# Autodesk Inventor assembly: EncoderAssembly_MIR1
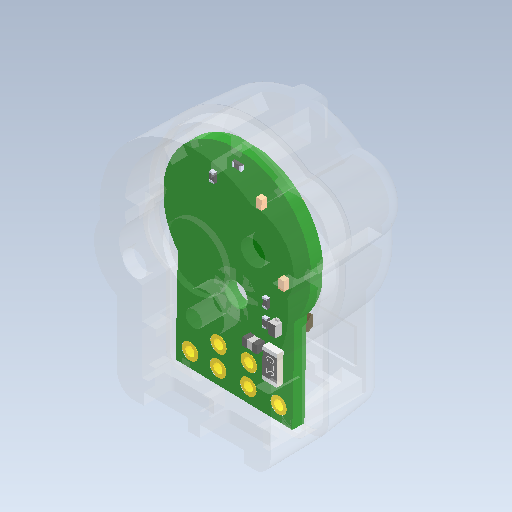
[picture p0: Inventor's stored thumbnail of the model, 512x512]
Saved by Autodesk Inventor 2020 (Build 240168000, 168)
## iProperties
Created: 2021-02-20
Part Number: EncoderAssembly_MIR1
Document SubType Name: Assembly
Designer: turnm
Author: turnm
## Documents named in this file (3)
- C:\Users\turnm\Documents\GrabCAD\Infinite Recharge 2020\Build season\EncoderCAD\EncoderAssembly_MIR1.iam
- C:\Users\turnm\Downloads\Cancoder_CAD\Housing_MIR1.ipt
- C:\Users\turnm\Downloads\Cancoder_CAD\PCB Assembly_MIR1.ipt
## Components (2 placed, 2 different names)
1. Housing_MIR1:1 — Flush:1, Mate:1
2. PCB Assembly_MIR1:1 — Flush:1, Mate:1
## Relationships (2: Flush 1, Mate 1)
- Flush:1 (7.112 mm): Housing_MIR1:1 ↔ PCB Assembly_MIR1:1
- Mate:1: Housing_MIR1:1 ↔ PCB Assembly_MIR1:1
